# Autodesk Inventor assembly: Belt_clamp_mirrored_print
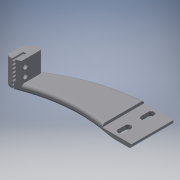
[picture p0: Inventor's stored thumbnail of the model, 180x180]
Saved by Autodesk Inventor 2019.3 (Build 233278000, 278)
## iProperties
Created: 2020-09-10
Part Number: Belt_clamp_mirrored_print
Material: Generisch
Document SubType Name: Assembly
Designer: Nicolas Frick
Author: Nicolas Frick
## Documents named in this file (2)
- C:\Users\Nicolas Frick\Sync\OneDrive\airhockeybot\mechanical_design\common_cad_parts\print_models\upper\Belt_clamp_mirrored_print.iam
- C:\Users\Nicolas Frick\Sync\OneDrive\airhockeybot\mechanical_design\inventor\Belt_clamp_mirrored.ipt
## Components (1 placed, 1 different names)
1. Belt_clamp_mirrored:1 — Passend:1, Passend:2, Passend:3
## Relationships (3: Mate 3)
- Passend:1 [Mate]: Belt_clamp_mirrored:1
- Passend:2 [Mate]: Belt_clamp_mirrored:1
- Passend:3 [Mate]: Belt_clamp_mirrored:1
